# Autodesk Inventor assembly: calle
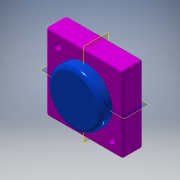
[picture p0: Inventor's stored thumbnail of the model, 180x180]
Saved by Autodesk Inventor 2019 (Build 230136000, 136)
## iProperties
Created: 2019-03-18
Part Number: calle
Document SubType Name: Assembly
Designer: franc
Author: franc
## Documents named in this file (3)
- C:\Users\franc\Desktop\EsialRobotik\Mecanique\composants\Profile\calle.iam
- C:\Users\franc\Desktop\EsialRobotik\Mecanique\composants\Profile\calle-patin.ipt
- C:\Users\franc\Desktop\EsialRobotik\Mecanique\composants\Profile\patin-teflon-24x5.ipt
## Components (2 placed, 2 different names)
1. calle-patin:1 — Placage:1, Affleurement:1, Affleurement:2
2. patin-teflon-24x5:1 — Placage:1, Placage:2, Placage:3
## Relationships (5: Mate 3, Flush 2)
- Placage:1 [Mate]: calle-patin:1 ↔ patin-teflon-24x5:1
- Affleurement:1 [Flush] (-17 mm): calle-patin:1
- Affleurement:2 [Flush] (-16.5 mm): calle-patin:1
- Placage:2 [Mate]: patin-teflon-24x5:1
- Placage:3 [Mate]: patin-teflon-24x5:1
